# Autodesk Inventor assembly: Aerosky MC4230 630KV
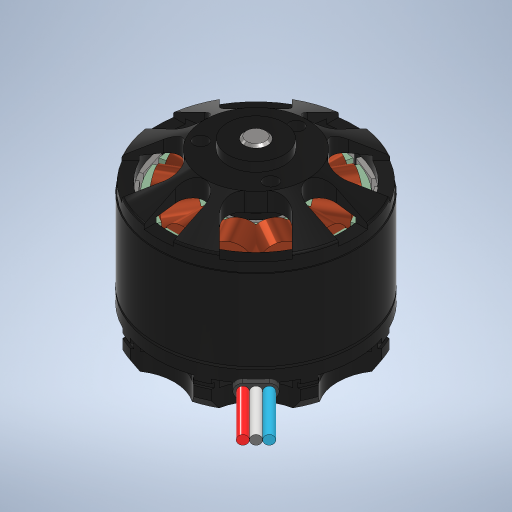
[picture p0: Inventor's stored thumbnail of the model, 512x512]
Saved by Autodesk Inventor 2023.2 (Build 272271000, 271)
## iProperties
Created: 2022-07-25
Part Number: Aerosky MC4230 630KV
Document SubType Name: Assembly
Designer: Nathan Cai
Mass: 140 g
Surface Area: 368.046 cm^2
Volume: 32.0745 cm^3
Density: 4.36483 g/cm^3
Author: Nathan Cai
## Documents named in this file (3)
- E:\Documents\Inventor\Moon Cake V0.13\Aerosky MC4230 630KV\Aerosky MC4230 630KV.iam
- E:\Documents\Inventor\Moon Cake V0.13\Aerosky MC4230 630KV\CAN.iam
- E:\Documents\Inventor\Moon Cake V0.13\Aerosky MC4230 630KV\BASE.iam
## Components (2 placed, 2 different names)
1. CAN:1 [sub-assembly] — Mate:1, Mate:2
2. BASE:1 [sub-assembly] — Mate:1, Mate:2
## Relationships (2: Mate 2)
- Mate:1: CAN:1 ↔ BASE:1
- Mate:2: CAN:1 ↔ BASE:1
